# Autodesk Inventor assembly: CycloidalDrive2
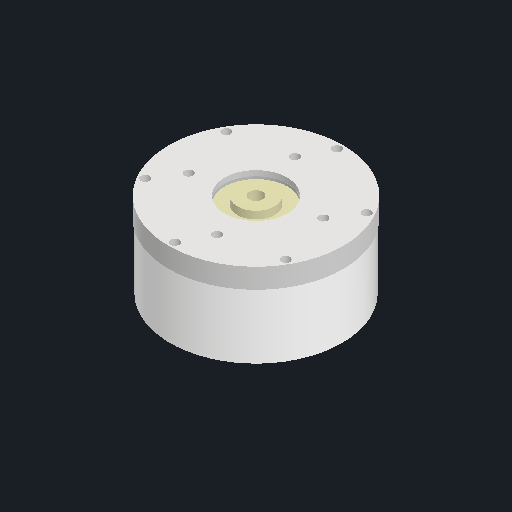
[picture p0: Inventor's stored thumbnail of the model, 512x512]
Saved by Autodesk Inventor 2022 (Build 260153000, 153)
## iProperties
Created: 2022-10-07
Part Number: CycloidalDrive2
Document SubType Name: Assembly
Designer: MicnedSQ
Author: MicnedSQ
## Documents named in this file (7)
- C:\Users\MicnedSQ\Desktop\RobotArmV1\RotatingBase\CycloidalDrive\CycloidalDrive2.iam
- C:\Users\MicnedSQ\Desktop\RobotArmV1\RotatingBase\CycloidalDrive\Bottom.ipt
- C:\Users\MicnedSQ\Desktop\RobotArmV1\RotatingBase\CycloidalDrive\OutputShaft.iam
- C:\Users\MicnedSQ\Desktop\RobotArmV1\RotatingBase\CycloidalDrive\CycloidalDisc.ipt
- C:\Users\MicnedSQ\Desktop\RobotArmV1\RotatingBase\CycloidalDrive\InputShaft.iam
- C:\Users\MicnedSQ\Desktop\RobotArmV1\Bearing 25x32x4\AIS2021\SKF_W 61705-2RS1.iam
- C:\Users\MicnedSQ\Desktop\RobotArmV1\RotatingBase\CycloidalDrive\Top.ipt
## Components (8 placed, 6 different names)
1. Bottom:1 — Obrotowe:1, Rotational:7
2. OutputShaft:1 [sub-assembly] — Obrotowe:1, Rotational:5
3. CycloidalDisc:1 — Rotational:6
4. InputShaft:1 [sub-assembly] — Rotational:2, Rotational:3, Rotational:4
5. SKF_W 61705-2RS1:1 [sub-assembly] — Rotational:2
6. SKF_W 61705-2RS1:2 [sub-assembly] — Rotational:4, Rotational:5
7. SKF_W 61705-2RS1:3 [sub-assembly] — Rotational:3, Rotational:6
8. Top:1 — Rotational:7
## Relationships (7: RevoluteJoint 7)
- Obrotowe:1 [RevoluteJoint]: Bottom:1 ↔ OutputShaft:1
- Rotational:2 [RevoluteJoint]: InputShaft:1 ↔ SKF_W 61705-2RS1:1
- Rotational:3 [RevoluteJoint]: InputShaft:1 ↔ SKF_W 61705-2RS1:3
- Rotational:4 [RevoluteJoint]: InputShaft:1 ↔ SKF_W 61705-2RS1:2
- Rotational:5 [RevoluteJoint]: OutputShaft:1 ↔ SKF_W 61705-2RS1:2
- Rotational:6 [RevoluteJoint]: CycloidalDisc:1 ↔ SKF_W 61705-2RS1:3
- Rotational:7 [RevoluteJoint]: Bottom:1 ↔ Top:1
